# Autodesk Inventor assembly: sub sytem part 1
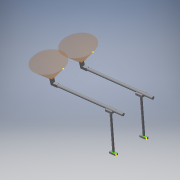
[picture p0: Inventor's stored thumbnail of the model, 180x180]
Saved by Autodesk Inventor 2019 (Build 230136000, 136)
## iProperties
Created: 2020-05-09
Part Number: sub sytem part 1
Document SubType Name: Assembly
Designer: Adityan Matthew
Author: Adityan Matthew
## Documents named in this file (6)
- D:\sub sytem part 1.iam
- D:\expopipe_CPY dS.ipt
- D:\expofunl2 dS.ipt
- D:\elbow3_CPY_CPY dS.ipt
- D:\base.ipt
- D:\sub system 1 base.ipt
## Components (10 placed, 5 different names)
1. expopipe_CPY dS:1 — Rigid:1, Mate:1
2. expofunl2 dS:1 — Rigid:2
3. elbow3_CPY_CPY dS:1 — Rigid:1, Rigid:2
4. base:1 — Rigid:3
5. sub system 1 base:1 — Mate:1, Rigid:3
6. expopipe_CPY dS:2
7. expofunl2 dS:2
8. elbow3_CPY_CPY dS:2
9. base:2
10. sub system 1 base:2
## Relationships (8: WeldJoint 6, Mate 2)
- Rigid:1 [WeldJoint]: expopipe_CPY dS:1 ↔ elbow3_CPY_CPY dS:1
- Rigid:2 [WeldJoint]: expofunl2 dS:1 ↔ elbow3_CPY_CPY dS:1
- Mate:1: expopipe_CPY dS:1 ↔ sub system 1 base:1
- Rigid:3 [WeldJoint]: base:1 ↔ sub system 1 base:1
- [WeldJoint]: expopipe_CPY dS:2 ↔ elbow3_CPY_CPY dS:2
- [WeldJoint]: expofunl2 dS:2 ↔ elbow3_CPY_CPY dS:2
- [Mate]: expopipe_CPY dS:2 ↔ sub system 1 base:2
- [WeldJoint]: base:2 ↔ sub system 1 base:2
## Named parameters: d4_d2 = 0 mm, d5_d3 = 0 mm, d6_d0 = 0 mm, d7_d1 = 0 mm
